# Autodesk Inventor assembly: proteox_fridge
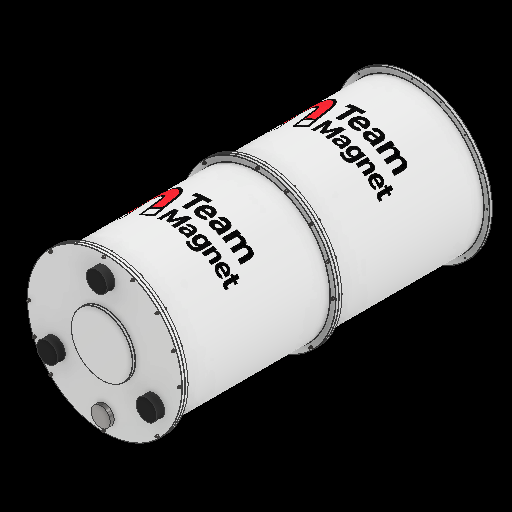
[picture p0: Inventor's stored thumbnail of the model, 512x512]
Saved by Autodesk Inventor 2026.1 (Build 301233000, 233)
## iProperties
Created: 2025-09-17
Part Number: proteox_fridge
Document SubType Name: Assembly
Designer: drago
Author: drago
## Documents named in this file (6)
- C:\Users\drago\Desktop\_QIST4500_Multidisciplinary_Team_Project\Proteox MX magnet positioner CAD\magnet_positioner_cad_design\proteox_mx_fridge\proteox_fridge.iam
- C:\Users\drago\Desktop\_QIST4500_Multidisciplinary_Team_Project\Proteox MX magnet positioner CAD\magnet_positioner_cad_design\proteox_mx_fridge\proteox_tube.ipt
- C:\Users\drago\Desktop\_QIST4500_Multidisciplinary_Team_Project\Proteox MX magnet positioner CAD\magnet_positioner_cad_design\proteox_mx_fridge\proteox_bottom_lid.ipt
- C:\Users\drago\Documents\Inventor\Content Center Files\R2026\en-US\ISO 7089\ISO 7089 - 5 - 140 HV(1).ipt
- C:\Users\drago\Documents\Inventor\Content Center Files\R2026\en-US\ISO 4762(2)\ISO 4762 - M5 x 35ISO.ipt
- C:\Users\drago\Documents\Inventor\Content Center Files\R2026\en-US\ISO 4032(2)\ISO 4032 - M5 - ISO.ipt
## Components (91 placed, 5 different names)
1. proteox_tube:1 — Mate:1, Mate:2, Mate:5, Mate:39, Mate:40, Mate:41, Mate:47, Mate:48, Mate:49, Mate:51, Mate:52, Mate:53, Mate:55, Mate:56, Mate:57
2. proteox_tube:2 — Mate:3, Angle:2, Mate:5, Mate:6, Mate:42, Mate:43, Mate:44, Mate:45, Mate:50, Mate:54, Mate:58, Mate:59, Mate:60, Mate:61, Mate:63, Mate:64, Mate:65, Mate:67, Mate:68, Mate:69
3. proteox_bottom_lid:1 — Mate:4, Angle:1, Mate:6, Mate:46, Mate:62, Mate:66, Mate:70
4. ISO 7089 5:33 — Mate:47, Mate:48, Insert:5
5. ISO 4762 M5 x 35:17 — Insert:5
6. ISO 7089 5:34 — Mate:49, Mate:50, Insert:6
7. ISO 4032 M5:17 — Insert:6
8. ISO 7089 5:35 — Mate:51, Mate:52, Insert:7
9. ISO 4762 M5 x 35:18 — Insert:7
10. ISO 7089 5:36 — Mate:53, Mate:54, Insert:8
11. ISO 4032 M5:18 — Insert:8
12. ISO 7089 5:37 — Mate:55, Mate:56, Insert:9
13. ISO 4762 M5 x 35:19 — Insert:9
14. ISO 7089 5:38 — Mate:57, Mate:58, Insert:10
15. ISO 4032 M5:19 — Insert:10
16. ISO 7089 5:39 — Mate:59, Mate:60, Insert:11
17. ISO 4762 M5 x 35:20 — Insert:11
18. ISO 7089 5:40 — Mate:61, Mate:62, Insert:12
19. ISO 4032 M5:20 — Insert:12
20. ISO 7089 5:41 — Mate:63, Mate:64, Insert:13
21. ISO 4762 M5 x 35:21 — Insert:13
22. ISO 7089 5:42 — Mate:65, Mate:66, Insert:14
23. ISO 4032 M5:21 — Insert:14
24. ISO 7089 5:43 — Mate:67, Mate:68, Insert:15
25. ISO 4762 M5 x 35:22 — Insert:15
26. ISO 7089 5:44 — Mate:69, Mate:70, Insert:16
27. ISO 4032 M5:22 — Insert:16
28. ISO 4762 M5 x 35:1 — Insert:1
29. ISO 7089 5:1 — Mate:39, Mate:40, Insert:1
30. ISO 7089 5:2 — Mate:41, Mate:42, Insert:2
31. ISO 4032 M5:1 — Insert:2
32. ISO 4762 M5 x 35:2
33. ISO 7089 5:3
34. ISO 7089 5:4
35. ISO 4032 M5:2
36. ISO 4762 M5 x 35:3
37. ISO 7089 5:5
38. ISO 7089 5:6
39. ISO 4032 M5:3
40. ISO 4762 M5 x 35:4
41. ISO 7089 5:7
42. ISO 7089 5:8
43. ISO 4032 M5:4
44. ISO 4762 M5 x 35:5
45. ISO 7089 5:9
46. ISO 7089 5:10
47. ISO 4032 M5:5
48. ISO 4762 M5 x 35:6
49. ISO 7089 5:11
50. ISO 7089 5:12
51. ISO 4032 M5:6
52. ISO 4762 M5 x 35:7
53. ISO 7089 5:13
54. ISO 7089 5:14
55. ISO 4032 M5:7
56. ISO 4762 M5 x 35:8
57. ISO 7089 5:15
58. ISO 7089 5:16
59. ISO 4032 M5:8
60. ISO 4762 M5 x 35:9 — Insert:3
61. ISO 7089 5:17 — Mate:43, Mate:44, Insert:3
62. ISO 7089 5:18 — Mate:45, Mate:46, Insert:4
63. ISO 4032 M5:9 — Insert:4
64. ISO 4762 M5 x 35:10
65. ISO 7089 5:19
66. ISO 7089 5:20
67. ISO 4032 M5:10
68. ISO 4762 M5 x 35:11
69. ISO 7089 5:21
70. ISO 7089 5:22
71. ISO 4032 M5:11
72. ISO 4762 M5 x 35:12
73. ISO 7089 5:23
74. ISO 7089 5:24
75. ISO 4032 M5:12
76. ISO 4762 M5 x 35:13
77. ISO 7089 5:25
78. ISO 7089 5:26
79. ISO 4032 M5:13
80. ISO 4762 M5 x 35:14
81. ISO 7089 5:27
82. ISO 7089 5:28
83. ISO 4032 M5:14
84. ISO 4762 M5 x 35:15
85. ISO 7089 5:29
86. ISO 7089 5:30
87. ISO 4032 M5:15
88. ISO 4762 M5 x 35:16
89. ISO 7089 5:31
90. ISO 7089 5:32
91. ISO 4032 M5:16
## Component patterns: (8 elements, first: ISO 4762 M5 x 35:1 + ISO 7089 5:1 + ISO 7089 5:2 + ISO 4032 M5:1), (8 elements, first: ISO 4762 M5 x 35:9 + ISO 7089 5:17 + ISO 7089 5:18 + ISO 4032 M5:9)
## Relationships (56: Mate 38, Insert 16, Angle 2)
- Mate:1: proteox_tube:1
- Mate:2: proteox_tube:1
- Mate:3: proteox_tube:2
- Mate:4: proteox_bottom_lid:1
- Angle:1 (0 deg): proteox_bottom_lid:1
- Angle:2 (0 deg): proteox_tube:2
- Mate:5: proteox_tube:1 ↔ proteox_tube:2
- Mate:6: proteox_tube:2 ↔ proteox_bottom_lid:1
- Mate:39: proteox_tube:1 ↔ ISO 7089 5:1
- Mate:40: proteox_tube:1 ↔ ISO 7089 5:1
- Insert:1: ISO 4762 M5 x 35:1 ↔ ISO 7089 5:1
- Mate:41: proteox_tube:1 ↔ ISO 7089 5:2
- Mate:42: proteox_tube:2 ↔ ISO 7089 5:2
- Insert:2: ISO 7089 5:2 ↔ ISO 4032 M5:1
- Mate:43: proteox_tube:2 ↔ ISO 7089 5:17
- Mate:44: proteox_tube:2 ↔ ISO 7089 5:17
- Insert:3: ISO 4762 M5 x 35:9 ↔ ISO 7089 5:17
- Mate:45: proteox_tube:2 ↔ ISO 7089 5:18
- Mate:46: proteox_bottom_lid:1 ↔ ISO 7089 5:18
- Insert:4: ISO 7089 5:18 ↔ ISO 4032 M5:9
- Mate:47: proteox_tube:1 ↔ ISO 7089 5:33
- Mate:48: proteox_tube:1 ↔ ISO 7089 5:33
- Insert:5: ISO 7089 5:33 ↔ ISO 4762 M5 x 35:17
- Mate:49: proteox_tube:1 ↔ ISO 7089 5:34
- Mate:50: proteox_tube:2 ↔ ISO 7089 5:34
- Insert:6: ISO 7089 5:34 ↔ ISO 4032 M5:17
- Mate:51: proteox_tube:1 ↔ ISO 7089 5:35
- Mate:52: proteox_tube:1 ↔ ISO 7089 5:35
- Insert:7: ISO 7089 5:35 ↔ ISO 4762 M5 x 35:18
- Mate:53: proteox_tube:1 ↔ ISO 7089 5:36
- Mate:54: proteox_tube:2 ↔ ISO 7089 5:36
- Insert:8: ISO 7089 5:36 ↔ ISO 4032 M5:18
- Mate:55: proteox_tube:1 ↔ ISO 7089 5:37
- Mate:56: proteox_tube:1 ↔ ISO 7089 5:37
- Insert:9: ISO 7089 5:37 ↔ ISO 4762 M5 x 35:19
- Mate:57: proteox_tube:1 ↔ ISO 7089 5:38
- Mate:58: proteox_tube:2 ↔ ISO 7089 5:38
- Insert:10: ISO 7089 5:38 ↔ ISO 4032 M5:19
- Mate:59: proteox_tube:2 ↔ ISO 7089 5:39
- Mate:60: proteox_tube:2 ↔ ISO 7089 5:39
- Insert:11: ISO 7089 5:39 ↔ ISO 4762 M5 x 35:20
- Mate:61: proteox_tube:2 ↔ ISO 7089 5:40
- Mate:62: proteox_bottom_lid:1 ↔ ISO 7089 5:40
- Insert:12: ISO 7089 5:40 ↔ ISO 4032 M5:20
- Mate:63: proteox_tube:2 ↔ ISO 7089 5:41
- Mate:64: proteox_tube:2 ↔ ISO 7089 5:41
- Insert:13: ISO 7089 5:41 ↔ ISO 4762 M5 x 35:21
- Mate:65: proteox_tube:2 ↔ ISO 7089 5:42
- Mate:66: proteox_bottom_lid:1 ↔ ISO 7089 5:42
- Insert:14: ISO 7089 5:42 ↔ ISO 4032 M5:21
- Mate:67: proteox_tube:2 ↔ ISO 7089 5:43
- Mate:68: proteox_tube:2 ↔ ISO 7089 5:43
- Insert:15: ISO 7089 5:43 ↔ ISO 4762 M5 x 35:22
- Mate:69: proteox_tube:2 ↔ ISO 7089 5:44
- Mate:70: proteox_bottom_lid:1 ↔ ISO 7089 5:44
- Insert:16: ISO 7089 5:44 ↔ ISO 4032 M5:22
